# Autodesk Inventor assembly: Assembly
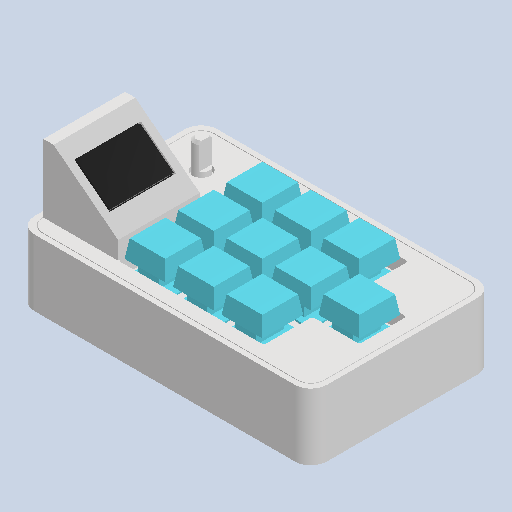
[picture p0: Inventor's stored thumbnail of the model, 512x512]
Saved by Autodesk Inventor 2025.2 (Build 292293000, 293)
## iProperties
Created: 2024-03-12
Part Number: Assembly
Document SubType Name: Assembly
Designer: mirun
Author: mirun
## Documents named in this file (10)
- C:\Users\mirewn\Documents\GitHub\Macropad\Assembly.iam
- C:\Users\mirewn\Documents\GitHub\Macropad\top.ipt
- C:\Users\mirewn\Documents\GitHub\Macropad\switch.ipt
- C:\Users\mirewn\Documents\GitHub\Macropad\Screen.ipt
- C:\Users\mirewn\Documents\GitHub\Macropad\bottom.ipt
- C:\Users\mirewn\Documents\GitHub\Macropad\usb.ipt
- C:\Users\mirewn\Documents\GitHub\Macropad\Battery.ipt
- C:\Users\mirewn\Documents\GitHub\Macropad\thing.ipt
- C:\Users\mirewn\Documents\Inventor\Content Center Files\R2025\en-US\DIN 7985 (H)\DIN 7985 (H) - M3x20-H.ipt
- C:\Users\mirewn\Documents\GitHub\Macropad\rotary.ipt
## Components (21 placed, 9 different names)
1. top:1 — Mate:1, Mate:2, Mate:3, Mate:4, Mate:5, Mate:6, Mate:7, Mate:8, Mate:9, Mate:10, Mate:11, Mate:12, Mate:13, Mate:22, Mate:23
2. switch:2 — Mate:4, Mate:5, Mate:6
3. Screen:1 — Mate:7, Mate:8, Mate:9, Mate:10
4. bottom:1 — Mate:11, Mate:12, Mate:13, Mate:14, Mate:15, Tangent:1, Mate:16, Mate:17, Mate:18, Mate:19, Mate:20, Mate:21, Insert:1, Insert:2, Insert:3, Insert:4
5. usb:1 — Mate:14, Mate:15, Tangent:1
6. Battery:1 — Mate:16, Mate:17, Mate:18
7. thing:1 — Mate:19, Mate:20, Mate:21
8. DIN 7985 (H) M3x20-H:1 — Insert:1
9. DIN 7985 (H) M3x20-H:2 — Insert:2
10. DIN 7985 (H) M3x20-H:3 — Insert:3
11. DIN 7985 (H) M3x20-H:4 — Insert:4
12. rotary:1 — Mate:22, Mate:23
13. switch:1 — Mate:1, Mate:2, Mate:3
14. switch:3
15. switch:4
16. switch:5
17. switch:6
18. switch:7
19. switch:8
20. switch:9
21. switch:10
## Component patterns: (9 elements, first: switch:1)
## Relationships (28: Mate 23, Insert 4, Tangent 1)
- Mate:1: top:1 ↔ switch:1
- Mate:2 (0.25 mm): top:1 ↔ switch:1
- Mate:3 (0.25 mm): top:1 ↔ switch:1
- Mate:4: top:1 ↔ switch:2
- Mate:5 (0.25 mm): top:1 ↔ switch:2
- Mate:6 (0.25 mm): top:1 ↔ switch:2
- Mate:7: top:1 ↔ Screen:1
- Mate:8 (0.5 mm): top:1 ↔ Screen:1
- Mate:9 (0.5 mm): top:1 ↔ Screen:1
- Mate:10: top:1 ↔ Screen:1
- Mate:11 (0.25 mm): top:1 ↔ bottom:1
- Mate:12 (0.25 mm): top:1 ↔ bottom:1
- Mate:13 (-0.25 mm): top:1 ↔ bottom:1
- Mate:14: bottom:1 ↔ usb:1
- Mate:15: bottom:1 ↔ usb:1
- Tangent:1 (7.25 mm): bottom:1 ↔ usb:1
- Mate:16: bottom:1 ↔ Battery:1
- Mate:17 (1 mm): bottom:1 ↔ Battery:1
- Mate:18 (1 mm): bottom:1 ↔ Battery:1
- Mate:19 (0.25 mm): bottom:1 ↔ thing:1
- Mate:20 (0.25 mm): bottom:1 ↔ thing:1
- Mate:21 (0.25 mm): bottom:1 ↔ thing:1
- Insert:1: bottom:1 ↔ DIN 7985 (H) M3x20-H:1
- Insert:2: bottom:1 ↔ DIN 7985 (H) M3x20-H:2
- Insert:3: bottom:1 ↔ DIN 7985 (H) M3x20-H:3
- Insert:4: bottom:1 ↔ DIN 7985 (H) M3x20-H:4
- Mate:22: top:1 ↔ rotary:1
- Mate:23 (1 mm): top:1 ↔ rotary:1
